# Autodesk Inventor assembly: Assembly2
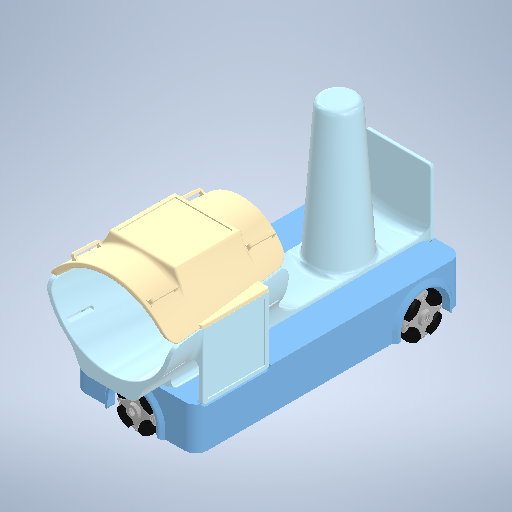
[picture p0: Inventor's stored thumbnail of the model, 512x512]
Saved by Autodesk Inventor 2025 (Build 290162000, 162)
## iProperties
Created: 2024-06-13
Part Number: Assembly2
Document SubType Name: Assembly
Designer: Pintu
Author: Pintu
## Documents named in this file (10)
- D:\CMC\my_inventor\ArmBo_v2\wearable\Assembly2.iam
- D:\CMC\my_inventor\ArmBo_v2\wearable\wearable.ipt
- D:\CMC\my_inventor\ArmBo_v2\wearable\aruco_top_marker.ipt
- D:\CMC\my_inventor\ArmBo_v2\wearable\new_base_old.ipt
- D:\CMC\my_inventor\ArmBo_v2\wearable\new_base.ipt
- D:\CMC\my_inventor\ArmBo_v2\wheels\omniwheel_38mm\omniwheel_38mm\wheel_38mm_assembly.iam
- D:\CMC\my_inventor\ArmBo_v2\wheels\omniwheel_38mm\omniwheel_38mm\wheel_holder.ipt
- C:\Users\Pintu\Documents\Inventor\Content Center Files\R2025\en-US\ISO 4762(2)\ISO 4762 - M3 x 30ISO.ipt
- C:\Users\Pintu\Documents\Inventor\Content Center Files\R2025\en-US\ISO 7089\ISO 7089 - 3 - 140 HV(1).ipt
- C:\Users\Pintu\Documents\Inventor\Content Center Files\R2025\en-US\ISO 4032(2)\ISO 4032 - M3 - ISO.ipt
## Components (16 placed, 9 different names)
1. wearable:1 — Flush:3, Flush:4, Flush:5, Mate:2
2. aruco_top_marker:1
3. new_base_old:1 — Flush:3
4. new_base:1 — Flush:4, Flush:5, Mate:2, Mate:6, Mate:7, Mate:8, Mate:9, Mate:12, Mate:13, Mate:18, Mate:22
5. wheel_38mm_assembly:1 [sub-assembly] — Mate:10
6. wheel_38mm_assembly:2 [sub-assembly] — Mate:14
7. wheel_38mm_assembly:3 [sub-assembly] — Mate:11
8. wheel_holder:1 — Mate:8, Mate:9, Mate:11
9. wheel_holder:2 — Mate:6, Mate:7, Mate:10, Mate:15, Mate:16, Mate:17, Mate:19, Mate:20, Mate:21
10. wheel_holder:3 — Mate:12, Mate:13, Mate:14
11. ISO 4762 M3 x 30:1 — Mate:15, Mate:16
12. ISO 7089 3:1 — Mate:17, Mate:18, Insert:1
13. ISO 4032 M3:1 — Insert:1
14. ISO 4762 M3 x 30:2 — Mate:19, Mate:20
15. ISO 7089 3:2 — Mate:21, Mate:22, Insert:2
16. ISO 4032 M3:2 — Insert:2
## Relationships (23: Mate 18, Flush 3, Insert 2)
- Flush:3: wearable:1 ↔ new_base_old:1
- Flush:4: wearable:1 ↔ new_base:1
- Flush:5 (25 mm): wearable:1 ↔ new_base:1
- Mate:2: wearable:1 ↔ new_base:1
- Mate:6: new_base:1 ↔ wheel_holder:2
- Mate:7: new_base:1 ↔ wheel_holder:2
- Mate:8: new_base:1 ↔ wheel_holder:1
- Mate:9: new_base:1 ↔ wheel_holder:1
- Mate:10: wheel_38mm_assembly:1 ↔ wheel_holder:2
- Mate:11: wheel_38mm_assembly:3 ↔ wheel_holder:1
- Mate:12: new_base:1 ↔ wheel_holder:3
- Mate:13: new_base:1 ↔ wheel_holder:3
- Mate:14: wheel_38mm_assembly:2 ↔ wheel_holder:3
- Mate:15: wheel_holder:2 ↔ ISO 4762 M3 x 30:1
- Mate:16: wheel_holder:2 ↔ ISO 4762 M3 x 30:1
- Mate:17: wheel_holder:2 ↔ ISO 7089 3:1
- Mate:18: new_base:1 ↔ ISO 7089 3:1
- Insert:1: ISO 7089 3:1 ↔ ISO 4032 M3:1
- Mate:19: wheel_holder:2 ↔ ISO 4762 M3 x 30:2
- Mate:20: wheel_holder:2 ↔ ISO 4762 M3 x 30:2
- Mate:21: wheel_holder:2 ↔ ISO 7089 3:2
- Mate:22: new_base:1 ↔ ISO 7089 3:2
- Insert:2: ISO 7089 3:2 ↔ ISO 4032 M3:2
